# Autodesk Inventor assembly: SimulationWheelAssembly
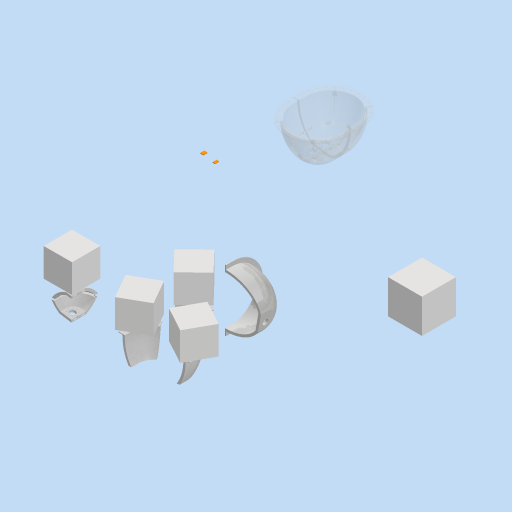
[picture p0: Inventor's stored thumbnail of the model, 512x512]
Saved by Autodesk Inventor 2023 (Build 270158000, 158)
## iProperties
Created: 2026-03-22
Part Number: SimulationWheelAssembly
Document SubType Name: Assembly
Designer: Nathann
Mass: 20175 g
Surface Area: 18221.2 cm^2
Volume: 20175 cm^3
Density: 1 g/cm^3
Author: Nathann
## Documents named in this file (22)
- C:\Users\Nathann\ClawdDrive\Objet3D\neodrive\neodrive-cad-ergonomic-v1\eggshellCorePrinted\SimulationWheelAssembly.iam
- C:\Users\Nathann\ClawdDrive\Objet3D\neodrive\neodrive-cad-ergonomic-v1\eggshellCorePrinted\prusaXL.ipt
- C:\Users\Nathann\ClawdDrive\Objet3D\neodrive\neodrive-cad-ergonomic-v1\eggshellCorePrinted\ImprimanteDario.ipt
- C:\Users\Nathann\ClawdDrive\Objet3D\neodrive\neodrive-cad-ergonomic-v1\eggshellCorePrinted\eggshellCorePrintedLeftA.ipt
- C:\Users\Nathann\ClawdDrive\Objet3D\neodrive\neodrive-cad-ergonomic-v1\eggshellCorePrinted\eggshellCorePrintedLeftE.ipt
- C:\Users\Nathann\ClawdDrive\Objet3D\neodrive\neodrive-cad-ergonomic-v1\eggshellCorePrinted\eggshellCorePrintedLeftF.ipt
- C:\Users\Nathann\ClawdDrive\Objet3D\neodrive\neodrive-cad-ergonomic-v1\eggshellCorePrinted\eggshellCorePrintedLeftG.ipt
- C:\Users\Nathann\ClawdDrive\Objet3D\neodrive\neodrive-cad-ergonomic-v1\eggshellCorePrinted\eggshellCorePrintedLeftH.ipt
- C:\Users\Nathann\ClawdDrive\Objet3D\neodrive\neodrive-cad-ergonomic-v1\eggshellCorePrinted\peg.ipt
- C:\Users\Nathann\ClawdDrive\Objet3D\neodrive\neodrive-cad-ergonomic-v1\eggshellCorePrinted\pegshort.ipt
- C:\Users\Nathann\ClawdDrive\Objet3D\neodrive\neodrive-cad-ergonomic-v1\eggshellCorePrinted\eggshellCorePrintedRightA.ipt
- C:\Users\Nathann\ClawdDrive\Objet3D\neodrive\neodrive-cad-ergonomic-v1\eggshellCorePrinted\eggshellCorePrintedRightE.ipt
- C:\Users\Nathann\ClawdDrive\Objet3D\neodrive\neodrive-cad-ergonomic-v1\eggshellCorePrinted\eggshellCorePrintedRightF.ipt
- C:\Users\Nathann\ClawdDrive\Objet3D\neodrive\neodrive-cad-ergonomic-v1\eggshellCorePrinted\eggshellCorePrintedRightG.ipt
- C:\Users\Nathann\ClawdDrive\Objet3D\neodrive\neodrive-cad-ergonomic-v1\eggshellCorePrinted\eggshellCorePrintedRightH.ipt
- C:\Users\Nathann\ClawdDrive\Objet3D\neodrive\neodrive-cad-ergonomic-v1\eggshellCorePrintedLeft.ipt
- C:\Users\Nathann\ClawdDrive\Objet3D\neodrive\neodrive-cad-ergonomic-v1\eggshellCorePrinted\SimulationWheelAssembly\AIP\FEA\fdktl59i8.fins
- C:\Users\Nathann\ClawdDrive\Objet3D\neodrive\neodrive-cad-ergonomic-v1\eggshellCorePrinted\SimulationWheelAssembly\AIP\FEA\fdktl59i8.fsat
- C:\Users\Nathann\ClawdDrive\Objet3D\neodrive\neodrive-cad-ergonomic-v1\eggshellCorePrinted\SimulationWheelAssembly\AIP\FEA\fdktl59j4.ftes
- C:\Users\Nathann\ClawdDrive\Objet3D\neodrive\neodrive-cad-ergonomic-v1\eggshellCorePrinted\SimulationWheelAssembly\AIP\FEA\fdktl59j4.fwiz
- C:\Users\Nathann\ClawdDrive\Objet3D\neodrive\neodrive-cad-ergonomic-v1\eggshellCorePrinted\SimulationWheelAssembly\AIP\FEA\fdktl59k0.fmsh
- C:\Users\Nathann\ClawdDrive\Objet3D\neodrive\neodrive-cad-ergonomic-v1\eggshellCorePrinted\SimulationWheelAssembly\AIP\FEA\fdktl59k1.fres
## Components (23 placed, 15 different names)
1. prusaXL:1
2. ImprimanteDario:1
3. eggshellCorePrintedLeftA:1 — Flush:1, Mate:8, Flush:2, Mate:9, Tangent:1, Flush:3, Mate:11
4. eggshellCorePrintedLeftE:1 — Flush:1, Mate:8, Flush:2, Mate:10, Flush:4, Tangent:2, Tangent:3
5. eggshellCorePrintedLeftF:1 — Mate:10, Flush:4, Tangent:2, Mate:12
6. eggshellCorePrintedLeftG:1 — Mate:11, Tangent:3, Mate:12
7. eggshellCorePrintedLeftH:1 — Mate:9, Tangent:1, Flush:3
8. eggshellCorePrintedLeftA:2
9. eggshellCorePrintedLeftE:2
10. eggshellCorePrintedLeftF:2
11. eggshellCorePrintedLeftG:2
12. eggshellCorePrintedLeftH:2
13. prusaXL:2
14. prusaXL:3
15. prusaXL:4
16. peg:1
17. pegshort:1
18. eggshellCorePrintedRightA:1 — Flush:5, Mate:13, Flush:6, Mate:16, Flush:8, Tangent:6, Mate:17
19. eggshellCorePrintedRightE:1 — Flush:5, Mate:13, Flush:6, Tangent:4, Flush:7, Mate:14, Tangent:5
20. eggshellCorePrintedRightF:1 — Tangent:4, Flush:7, Mate:14, Mate:15
21. eggshellCorePrintedRightG:1 — Mate:15, Tangent:5, Mate:16
22. eggshellCorePrintedRightH:1 — Flush:8, Tangent:6, Mate:17
23. eggshellCorePrintedLeft:1
## Relationships (24: Mate 10, Flush 8, Tangent 6)
- Flush:1: eggshellCorePrintedLeftA:1 ↔ eggshellCorePrintedLeftE:1
- Mate:8: eggshellCorePrintedLeftA:1 ↔ eggshellCorePrintedLeftE:1
- Flush:2: eggshellCorePrintedLeftA:1 ↔ eggshellCorePrintedLeftE:1
- Mate:9: eggshellCorePrintedLeftA:1 ↔ eggshellCorePrintedLeftH:1
- Tangent:1: eggshellCorePrintedLeftA:1 ↔ eggshellCorePrintedLeftH:1
- Flush:3: eggshellCorePrintedLeftA:1 ↔ eggshellCorePrintedLeftH:1
- Mate:10: eggshellCorePrintedLeftE:1 ↔ eggshellCorePrintedLeftF:1
- Flush:4: eggshellCorePrintedLeftE:1 ↔ eggshellCorePrintedLeftF:1
- Tangent:2: eggshellCorePrintedLeftE:1 ↔ eggshellCorePrintedLeftF:1
- Mate:11: eggshellCorePrintedLeftA:1 ↔ eggshellCorePrintedLeftG:1
- Tangent:3: eggshellCorePrintedLeftE:1 ↔ eggshellCorePrintedLeftG:1
- Mate:12: eggshellCorePrintedLeftF:1 ↔ eggshellCorePrintedLeftG:1
- Flush:5: eggshellCorePrintedRightA:1 ↔ eggshellCorePrintedRightE:1
- Mate:13: eggshellCorePrintedRightA:1 ↔ eggshellCorePrintedRightE:1
- Flush:6: eggshellCorePrintedRightA:1 ↔ eggshellCorePrintedRightE:1
- Tangent:4: eggshellCorePrintedRightE:1 ↔ eggshellCorePrintedRightF:1
- Flush:7: eggshellCorePrintedRightE:1 ↔ eggshellCorePrintedRightF:1
- Mate:14: eggshellCorePrintedRightE:1 ↔ eggshellCorePrintedRightF:1
- Mate:15: eggshellCorePrintedRightF:1 ↔ eggshellCorePrintedRightG:1
- Tangent:5: eggshellCorePrintedRightE:1 ↔ eggshellCorePrintedRightG:1
- Mate:16: eggshellCorePrintedRightA:1 ↔ eggshellCorePrintedRightG:1
- Flush:8: eggshellCorePrintedRightA:1 ↔ eggshellCorePrintedRightH:1
- Tangent:6: eggshellCorePrintedRightA:1 ↔ eggshellCorePrintedRightH:1
- Mate:17: eggshellCorePrintedRightA:1 ↔ eggshellCorePrintedRightH:1
## Named parameters: sa_0 = 300000, sa_1 = 0 mm, sa_2 = -700 mm, sa_3 = 0 mm, sa_4 = 300000
note: some values were not read from the file. Shown as the stored number, unit unknown: "sa_0", "sa_4".
